# Autodesk Inventor assembly: мёртвое колесо 25-26
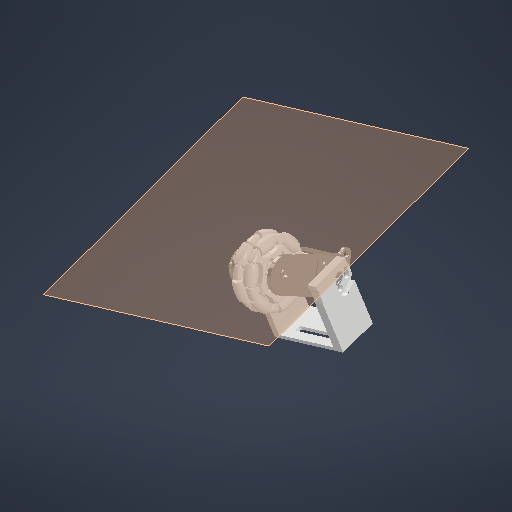
[picture p0: Inventor's stored thumbnail of the model, 512x512]
Saved by Autodesk Inventor 2025 (Build 290162000, 162)
## iProperties
Created: 2024-08-28
Part Number: мёртвое колесо 25-26
Document SubType Name: Assembly
Designer: Phantom
Author: Phantom
## Documents named in this file (7)
- C:\Users\Phantom\Desktop\Phantom16950\мёртвое колесо 25-26.iam
- C:\Users\Phantom\Desktop\Phantom16950\3110-0001-0001 assembly_MIR4.iam
- C:\Users\Phantom\Desktop\Phantom16950\1120-0003-0096_MIR1_MIR4.ipt
- C:\Users\Phantom\Desktop\Phantom16950\2915-0001-0003\2915-0001-0003_MIR2.ipt
- C:\Users\Phantom\Desktop\Phantom16950\1502-0006-0120\1502-0006-0120_MIR2.ipt
- C:\Users\Phantom\Desktop\Phantom16950\2800-0004-0020\2800-0004-0020_MIR2.ipt
- C:\Users\Phantom\Desktop\Phantom16950\2812-0004-0007\2812-0004-0007_MIR2.ipt
## Components (6 placed, 6 different names)
1. 3110-0001-0001 assembly_MIR4:1 [sub-assembly] — Совмещение:7
2. 1120-0003-0096_MIR1_MIR4:1 — Совмещение:1, Совмещение:3, Совмещение:2, Совмещение:6, Заподлицо:1, Совмещение:7
3. 2915-0001-0003_MIR2:1 — Совмещение:1
4. 1502-0006-0120_MIR2:1 — Совмещение:3, Совмещение:2, Совмещение:4
5. 2800-0004-0020_MIR2:1 — Совмещение:4, Совмещение:5
6. 2812-0004-0007_MIR2:1 — Совмещение:6, Совмещение:5
## Relationships (8: Mate 7, Flush 1)
- Совмещение:1 [Mate]: 1120-0003-0096_MIR1_MIR4:1 ↔ 2915-0001-0003_MIR2:1
- Совмещение:3 [Mate]: 1120-0003-0096_MIR1_MIR4:1 ↔ 1502-0006-0120_MIR2:1
- Совмещение:2 [Mate]: 1120-0003-0096_MIR1_MIR4:1 ↔ 1502-0006-0120_MIR2:1
- Совмещение:4 [Mate]: 1502-0006-0120_MIR2:1 ↔ 2800-0004-0020_MIR2:1
- Совмещение:6 [Mate]: 1120-0003-0096_MIR1_MIR4:1 ↔ 2812-0004-0007_MIR2:1
- Совмещение:5 [Mate]: 2800-0004-0020_MIR2:1 ↔ 2812-0004-0007_MIR2:1
- Заподлицо:1 [Flush] (40 mm): 1120-0003-0096_MIR1_MIR4:1
- Совмещение:7 [Mate]: 3110-0001-0001 assembly_MIR4:1 ↔ 1120-0003-0096_MIR1_MIR4:1
